# Autodesk Inventor assembly: FrontLink
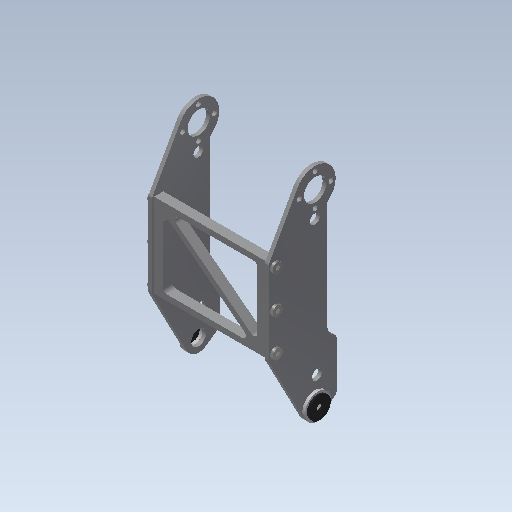
[picture p0: Inventor's stored thumbnail of the model, 512x512]
Saved by Autodesk Inventor 2020 (Build 240168000, 168)
## iProperties
Created: 2016-08-23
Part Number: FrontLink
Material: 一般
Document SubType Name: Assembly
Designer: hiro
Mass: 33.5175 g
Surface Area: 182.778 cm^2
Volume: 15.549 cm^3
Density: 2.15561 g/cm^3
Author: hiro
## Documents named in this file (6)
- C:\Users\Masato\Documents\Inventor\CIT Brains_Inventor\OpenPlatform_ver3_0\LowerBody\Link\FrontLink.iam
- C:\Users\Masato\Documents\Inventor\CIT Brains_Inventor\OpenPlatform_ver3_0\LowerBody\Link\FrontLink_diagonal.ipt
- C:\Users\Masato\Documents\Inventor\CIT Brains_Inventor\OpenPlatform_ver3_0\Ready_Made\UUW-0312-10BH.ipt
- C:\Users\Masato\Documents\Inventor\CIT Brains_Inventor\OpenPlatform_ver3_0\Ready_Made\Screw\M3-6.ipt
- C:\Users\Masato\Documents\Inventor\CIT Brains_Inventor\OpenPlatform_ver3_0\LowerBody\Link\FrontLink_frame.ipt
- C:\Users\Masato\Documents\Inventor\CIT Brains_Inventor\OpenPlatform_ver3_0\Ready_Made\TT-0814-15.ipt
## Components (13 placed, 5 different names)
1. FrontLink_diagonal:1 — 挿入:23, 挿入:24, 挿入:25, 挿入:30, 挿入:31, 挿入:32, フラッシュ:2, メイト:1
2. UUW-0312-10BH:1 — 挿入:38
3. UUW-0312-10BH:2 — 挿入:39
4. M3-6:1 — 挿入:26
5. M3-6:2 — 挿入:27
6. M3-6:3 — 挿入:28
7. M3-6:4 — 挿入:33
8. M3-6:5 — 挿入:35
9. M3-6:6 — 挿入:34
10. FrontLink_frame:1 — 挿入:23, 挿入:24, 挿入:25, 挿入:26, 挿入:27, 挿入:28, 挿入:36
11. FrontLink_frame:2 — 挿入:30, 挿入:31, 挿入:32, 挿入:33, 挿入:34, 挿入:35, フラッシュ:3, 挿入:37
12. TT-0814-15:1 — 挿入:36, 挿入:39
13. TT-0814-15:2 — 挿入:37, 挿入:38
## Relationships (19: Insert 16, Flush 2, Mate 1)
- 挿入:23 [Insert]: FrontLink_diagonal:1 ↔ FrontLink_frame:1
- 挿入:24 [Insert]: FrontLink_diagonal:1 ↔ FrontLink_frame:1
- 挿入:25 [Insert]: FrontLink_diagonal:1 ↔ FrontLink_frame:1
- 挿入:26 [Insert]: M3-6:1 ↔ FrontLink_frame:1
- 挿入:27 [Insert]: M3-6:2 ↔ FrontLink_frame:1
- 挿入:28 [Insert]: M3-6:3 ↔ FrontLink_frame:1
- 挿入:30 [Insert]: FrontLink_diagonal:1 ↔ FrontLink_frame:2
- 挿入:31 [Insert]: FrontLink_diagonal:1 ↔ FrontLink_frame:2
- 挿入:32 [Insert]: FrontLink_diagonal:1 ↔ FrontLink_frame:2
- 挿入:33 [Insert]: M3-6:4 ↔ FrontLink_frame:2
- 挿入:34 [Insert]: M3-6:6 ↔ FrontLink_frame:2
- 挿入:35 [Insert]: M3-6:5 ↔ FrontLink_frame:2
- フラッシュ:2 [Flush]: FrontLink_diagonal:1
- メイト:1 [Mate]: FrontLink_diagonal:1
- フラッシュ:3 [Flush]: FrontLink_frame:2
- 挿入:36 [Insert]: FrontLink_frame:1 ↔ TT-0814-15:1
- 挿入:37 [Insert]: FrontLink_frame:2 ↔ TT-0814-15:2
- 挿入:38 [Insert]: UUW-0312-10BH:1 ↔ TT-0814-15:2
- 挿入:39 [Insert]: UUW-0312-10BH:2 ↔ TT-0814-15:1
